# Autodesk Inventor assembly: __VK_Transferband
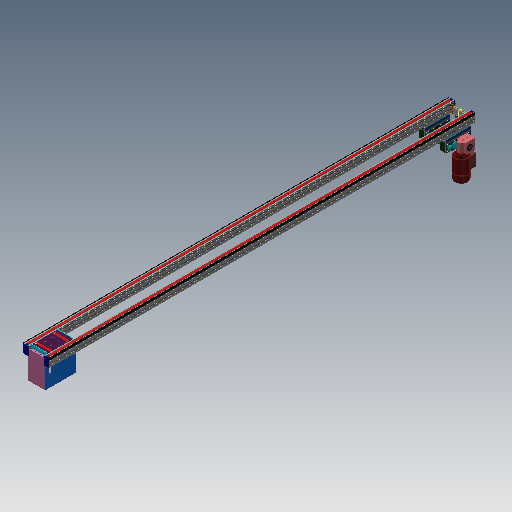
[picture p0: Inventor's stored thumbnail of the model, 512x512]
Saved by Autodesk Inventor 2019 (Build 230136000, 136)
## iProperties
Created: 2023-11-18
Part Number: __VK_Transferband
Material: Generisch
Document SubType Name: Assembly
Designer: RP
Author: RP
## Documents named in this file (5)
- C:\Users\RP\Documents\Inventor\Projekt_Angelspule\_Verkettung\__VK_Transferband.iam
- C:\Users\RP\Documents\Inventor\Projekt_Angelspule\_Verkettung\__VK_Quertransport.ipt
- C:\Users\RP\Documents\Inventor\Projekt_Angelspule\_Verkettung\__VK_Verbinder.ipt
- C:\Users\RP\Documents\Inventor\Projekt_Angelspule\_Verkettung\__VK_Antriebsmodul.ipt
- C:\Users\RP\Documents\Inventor\Projekt_Angelspule\_Verkettung\__VK_Seitenmodul.ipt
## Components (5 placed, 4 different names)
1. __VK_Verbinder:1 — Fluchtend:3, Passend:10
2. __VK_Seitenmodul:1 — Fluchtend:2, Passend:6, Passend:7, Passend:8, Fluchtend:5, Passend:11
3. __VK_Seitenmodul:2 — Fluchtend:1, Passend:8, Passend:9, Passend:10
4. __VK_Quertransport:1 — Fluchtend:4, Fluchtend:5
5. __VK_Antriebsmodul:1 — Passend:6, Passend:7, Passend:11
## Relationships (15: Mate 10, Flush 5)
- [Mate]: __VK_Verbinder:1 ↔ __VK_Seitenmodul:1
- [Mate]: __VK_Verbinder:1 ↔ __VK_Seitenmodul:2
- [Mate]: __VK_Verbinder:1 ↔ __VK_Seitenmodul:1
- [Mate]: __VK_Seitenmodul:2 ↔ __VK_Quertransport:1
- Fluchtend:1 [Flush]: __VK_Seitenmodul:2
- Fluchtend:2 [Flush]: __VK_Seitenmodul:1
- Passend:6 [Mate]: __VK_Seitenmodul:1 ↔ __VK_Antriebsmodul:1
- Passend:7 [Mate] (0.2 mm): __VK_Seitenmodul:1 ↔ __VK_Antriebsmodul:1
- Fluchtend:3 [Flush]: __VK_Verbinder:1
- Passend:8 [Mate]: __VK_Seitenmodul:1 ↔ __VK_Seitenmodul:2
- Passend:9 [Mate]: __VK_Seitenmodul:2
- Fluchtend:4 [Flush]: __VK_Quertransport:1
- Fluchtend:5 [Flush]: __VK_Seitenmodul:1 ↔ __VK_Quertransport:1
- Passend:10 [Mate]: __VK_Verbinder:1 ↔ __VK_Seitenmodul:2
- Passend:11 [Mate] (50 mm): __VK_Seitenmodul:1 ↔ __VK_Antriebsmodul:1
